# Autodesk Inventor assembly: Chassis assembly
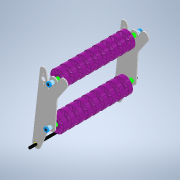
[picture p0: Inventor's stored thumbnail of the model, 180x180]
Saved by Autodesk Inventor 2022 (Build 260153000, 153)
## iProperties
Created: 2022-11-14
Part Number: Chassis assembly
Document SubType Name: Assembly
Designer: s135320
Author: s135320
## Documents named in this file (9)
- D:\Intake assembly.iam
- D:\STEP Files\Bearings\1-2inch Hex Bering\217-3875-STEP-20140818.ipt
- D:\STEP Files\Hardware\Shaft Collars\TTB Balanced Hex Collar\TTB-0013_Balanced Half Inch Hex Shaft Collar.ipt
- D:\Intake hex.ipt
- D:\intake-1.ipt
- D:\TTB-0058 5M 15t HTD ALUMINUM PULLEY.ipt
- D:\am-3480 4IN 500Hex Bore Compliant Wheel REV2.ipt
- D:\am-4541 Sushi Roller 500 Hex Bore.ipt
- D:\Intake base hex.ipt
## Components (56 placed, 8 different names)
1. TTB-0058 5M 15t HTD ALUMINUM PULLEY:3 — Mate:538, Mate:539, Mate:540, Mate:541
2. Intake base hex:1 — Mate:532, Mate:533, Mate:536, Mate:537
3. 217-3875-STEP-20140818:30 — Mate:528, Mate:529, Mate:536
4. 217-3875-STEP-20140818:31 — Mate:531, Mate:532, Mate:533, Mate:535
5. TTB-0013_Balanced Half Inch Hex Shaft Collar:15 — Mate:490, Mate:491, Mate:540
6. am-4541 Sushi Roller 500 Hex Bore:32 — Mate:492, Mate:493, Mate:501
7. TTB-0013_Balanced Half Inch Hex Shaft Collar:16 — Mate:497, Mate:498, Mate:499, Flush:22
8. 217-3875-STEP-20140818:25 — Mate:480, Mate:481, Mate:484, Mate:485, Mate:486, Mate:487, Mate:541
9. 217-3875-STEP-20140818:24 — Mate:482, Mate:483, Mate:499, Mate:511, Mate:512
10. am-4541 Sushi Roller 500 Hex Bore:2 — Mate:508, Mate:509, Mate:510
11. intake-1:3 — Mate:480, Mate:481, Mate:482, Mate:486, Mate:487, Mate:501, Mate:510, Mate:512, Mate:531, Mate:535
12. TTB-0013_Balanced Half Inch Hex Shaft Collar:13 — Mate:442, Mate:443, Flush:21, Mate:444
13. TTB-0013_Balanced Half Inch Hex Shaft Collar:12 — Flush:20, Mate:445, Mate:472
14. TTB-0058 5M 15t HTD ALUMINUM PULLEY:2 — Mate:436, Mate:437, Mate:438, Mate:444
15. TTB-0058 5M 15t HTD ALUMINUM PULLEY:1 — Mate:434, Mate:435, Mate:439, Mate:445
16. 217-3875-STEP-20140818:23 — Mate:433, Mate:439, Mate:469, Mate:472
17. 217-3875-STEP-20140818:22 — Mate:431, Mate:432, Mate:438, Mate:475
18. intake-1:2 — Mate:507, Mate:528, Mate:529, Mate:537
19. Intake hex:2 — Mate:433, Mate:434, Mate:435, Flush:20, Mate:469, Mate:484, Mate:485, Mate:490, Mate:491, Mate:502, Mate:503, Mate:504, Mate:505, Mate:508, Mate:509, Mate:538, Mate:539
20. Intake hex:1 — Mate:431, Mate:432, Mate:436, Mate:437, Mate:442, Mate:443, Flush:21, Mate:473, Mate:474, Mate:476, Mate:477, Mate:483, Mate:492, Mate:493, Mate:497, Mate:498, Mate:511, Flush:22
21. am-4541 Sushi Roller 500 Hex Bore:33 — Mate:502, Mate:503, Mate:506, Mate:507
22. am-3480 4IN 500Hex Bore Compliant Wheel REV2:33 — Mate:504, Mate:505, Mate:506
23. am-4541 Sushi Roller 500 Hex Bore:34
24. am-3480 4IN 500Hex Bore Compliant Wheel REV2:34
25. am-4541 Sushi Roller 500 Hex Bore:35
26. am-3480 4IN 500Hex Bore Compliant Wheel REV2:35
27. am-4541 Sushi Roller 500 Hex Bore:36
28. am-3480 4IN 500Hex Bore Compliant Wheel REV2:36
29. am-4541 Sushi Roller 500 Hex Bore:37
30. am-3480 4IN 500Hex Bore Compliant Wheel REV2:37
31. am-4541 Sushi Roller 500 Hex Bore:38
32. am-3480 4IN 500Hex Bore Compliant Wheel REV2:38
33. am-4541 Sushi Roller 500 Hex Bore:39
34. am-3480 4IN 500Hex Bore Compliant Wheel REV2:39
35. am-4541 Sushi Roller 500 Hex Bore:40
36. am-3480 4IN 500Hex Bore Compliant Wheel REV2:40
37. am-4541 Sushi Roller 500 Hex Bore:41
38. am-3480 4IN 500Hex Bore Compliant Wheel REV2:41
39. am-3480 4IN 500Hex Bore Compliant Wheel REV2:8 — Mate:476, Mate:477, Mate:478
40. am-4541 Sushi Roller 500 Hex Bore:23 — Mate:473, Mate:474, Mate:475, Mate:478
41. am-3480 4IN 500Hex Bore Compliant Wheel REV2:25
42. am-4541 Sushi Roller 500 Hex Bore:24
43. am-3480 4IN 500Hex Bore Compliant Wheel REV2:26
44. am-4541 Sushi Roller 500 Hex Bore:25
45. am-3480 4IN 500Hex Bore Compliant Wheel REV2:27
46. am-4541 Sushi Roller 500 Hex Bore:26
47. am-3480 4IN 500Hex Bore Compliant Wheel REV2:28
48. am-4541 Sushi Roller 500 Hex Bore:27
49. am-3480 4IN 500Hex Bore Compliant Wheel REV2:29
50. am-4541 Sushi Roller 500 Hex Bore:28
51. am-3480 4IN 500Hex Bore Compliant Wheel REV2:30
52. am-4541 Sushi Roller 500 Hex Bore:29
53. am-3480 4IN 500Hex Bore Compliant Wheel REV2:31
54. am-4541 Sushi Roller 500 Hex Bore:30
55. am-3480 4IN 500Hex Bore Compliant Wheel REV2:32
56. am-4541 Sushi Roller 500 Hex Bore:31
## Component patterns: (9 elements, first: am-4541 Sushi Roller 500 Hex Bore:33 + am-3480 4IN 500Hex Bore Compliant Wheel REV2:33), (9 elements, first: am-3480 4IN 500Hex Bore Compliant Wheel REV2:8 + am-4541 Sushi Roller 500 Hex Bore:23)
## Relationships (67: Mate 64, Flush 3)
- [Mate]: 217-3875-STEP-20140818:22 ↔ intake-1:2
- [Mate]: 217-3875-STEP-20140818:22 ↔ intake-1:2
- [Mate]: 217-3875-STEP-20140818:23 ↔ intake-1:2
- [Mate]: 217-3875-STEP-20140818:23 ↔ intake-1:2
- Mate:431: 217-3875-STEP-20140818:22 ↔ Intake hex:1
- Mate:432: 217-3875-STEP-20140818:22 ↔ Intake hex:1
- Mate:433: 217-3875-STEP-20140818:23 ↔ Intake hex:2
- Mate:434: TTB-0058 5M 15t HTD ALUMINUM PULLEY:1 ↔ Intake hex:2
- Mate:435: TTB-0058 5M 15t HTD ALUMINUM PULLEY:1 ↔ Intake hex:2
- Mate:436: TTB-0058 5M 15t HTD ALUMINUM PULLEY:2 ↔ Intake hex:1
- Mate:437: TTB-0058 5M 15t HTD ALUMINUM PULLEY:2 ↔ Intake hex:1
- Mate:438: TTB-0058 5M 15t HTD ALUMINUM PULLEY:2 ↔ 217-3875-STEP-20140818:22
- Mate:439: TTB-0058 5M 15t HTD ALUMINUM PULLEY:1 ↔ 217-3875-STEP-20140818:23
- Flush:20: TTB-0013_Balanced Half Inch Hex Shaft Collar:12 ↔ Intake hex:2
- Mate:442: TTB-0013_Balanced Half Inch Hex Shaft Collar:13 ↔ Intake hex:1
- Mate:443: TTB-0013_Balanced Half Inch Hex Shaft Collar:13 ↔ Intake hex:1
- Flush:21: TTB-0013_Balanced Half Inch Hex Shaft Collar:13 ↔ Intake hex:1
- Mate:444: TTB-0013_Balanced Half Inch Hex Shaft Collar:13 ↔ TTB-0058 5M 15t HTD ALUMINUM PULLEY:2
- Mate:445: TTB-0013_Balanced Half Inch Hex Shaft Collar:12 ↔ TTB-0058 5M 15t HTD ALUMINUM PULLEY:1
- Mate:469: 217-3875-STEP-20140818:23 ↔ Intake hex:2
- Mate:472: TTB-0013_Balanced Half Inch Hex Shaft Collar:12 ↔ 217-3875-STEP-20140818:23
- Mate:473: Intake hex:1 ↔ am-4541 Sushi Roller 500 Hex Bore:23
- Mate:474: Intake hex:1 ↔ am-4541 Sushi Roller 500 Hex Bore:23
- Mate:475: 217-3875-STEP-20140818:22 ↔ am-4541 Sushi Roller 500 Hex Bore:23
- Mate:476: Intake hex:1 ↔ am-3480 4IN 500Hex Bore Compliant Wheel REV2:8
- Mate:477: Intake hex:1 ↔ am-3480 4IN 500Hex Bore Compliant Wheel REV2:8
- Mate:478: am-3480 4IN 500Hex Bore Compliant Wheel REV2:8 ↔ am-4541 Sushi Roller 500 Hex Bore:23
- Mate:480: 217-3875-STEP-20140818:25 ↔ intake-1:3
- Mate:481: 217-3875-STEP-20140818:25 ↔ intake-1:3
- Mate:482: 217-3875-STEP-20140818:24 ↔ intake-1:3
- Mate:483: 217-3875-STEP-20140818:24 ↔ Intake hex:1
- Mate:484: 217-3875-STEP-20140818:25 ↔ Intake hex:2
- Mate:485: 217-3875-STEP-20140818:25 ↔ Intake hex:2
- Mate:486: 217-3875-STEP-20140818:25 ↔ intake-1:3
- Mate:487: 217-3875-STEP-20140818:25 ↔ intake-1:3
- Mate:490: TTB-0013_Balanced Half Inch Hex Shaft Collar:15 ↔ Intake hex:2
- Mate:491: TTB-0013_Balanced Half Inch Hex Shaft Collar:15 ↔ Intake hex:2
- Mate:492: am-4541 Sushi Roller 500 Hex Bore:32 ↔ Intake hex:1
- Mate:493: am-4541 Sushi Roller 500 Hex Bore:32 ↔ Intake hex:1
- Mate:497: TTB-0013_Balanced Half Inch Hex Shaft Collar:16 ↔ Intake hex:1
- Mate:498: TTB-0013_Balanced Half Inch Hex Shaft Collar:16 ↔ Intake hex:1
- Mate:499: TTB-0013_Balanced Half Inch Hex Shaft Collar:16 ↔ 217-3875-STEP-20140818:24
- Mate:501: am-4541 Sushi Roller 500 Hex Bore:32 ↔ intake-1:3
- Mate:502: Intake hex:2 ↔ am-4541 Sushi Roller 500 Hex Bore:33
- Mate:503: Intake hex:2 ↔ am-4541 Sushi Roller 500 Hex Bore:33
- Mate:504: Intake hex:2 ↔ am-3480 4IN 500Hex Bore Compliant Wheel REV2:33
- Mate:505: Intake hex:2 ↔ am-3480 4IN 500Hex Bore Compliant Wheel REV2:33
- Mate:506: am-4541 Sushi Roller 500 Hex Bore:33 ↔ am-3480 4IN 500Hex Bore Compliant Wheel REV2:33
- Mate:507: intake-1:2 ↔ am-4541 Sushi Roller 500 Hex Bore:33
- Mate:508: am-4541 Sushi Roller 500 Hex Bore:2 ↔ Intake hex:2
- Mate:509: am-4541 Sushi Roller 500 Hex Bore:2 ↔ Intake hex:2
- Mate:510: am-4541 Sushi Roller 500 Hex Bore:2 ↔ intake-1:3
- Mate:511: 217-3875-STEP-20140818:24 ↔ Intake hex:1
- Mate:512: 217-3875-STEP-20140818:24 ↔ intake-1:3
- Flush:22 (11.43 mm): TTB-0013_Balanced Half Inch Hex Shaft Collar:16 ↔ Intake hex:1
- Mate:528: 217-3875-STEP-20140818:30 ↔ intake-1:2
- Mate:529: 217-3875-STEP-20140818:30 ↔ intake-1:2
- Mate:531: 217-3875-STEP-20140818:31 ↔ intake-1:3
- Mate:532: Intake base hex:1 ↔ 217-3875-STEP-20140818:31
- Mate:533: Intake base hex:1 ↔ 217-3875-STEP-20140818:31
- Mate:535: 217-3875-STEP-20140818:31 ↔ intake-1:3
- Mate:536: Intake base hex:1 ↔ 217-3875-STEP-20140818:30
- Mate:537 (-50.8 mm): Intake base hex:1 ↔ intake-1:2
- Mate:538: TTB-0058 5M 15t HTD ALUMINUM PULLEY:3 ↔ Intake hex:2
- Mate:539: TTB-0058 5M 15t HTD ALUMINUM PULLEY:3 ↔ Intake hex:2
- Mate:540: TTB-0058 5M 15t HTD ALUMINUM PULLEY:3 ↔ TTB-0013_Balanced Half Inch Hex Shaft Collar:15
- Mate:541: TTB-0058 5M 15t HTD ALUMINUM PULLEY:3 ↔ 217-3875-STEP-20140818:25
## Named parameters: d465_d457 = 0 mm, d466_d458 = 0 mm, d467_d459 = 0 mm, d468_d460 = 0 mm
